# Autodesk Inventor assembly: Inverse belt reducer
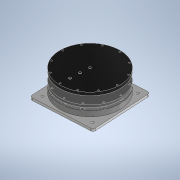
[picture p0: Inventor's stored thumbnail of the model, 180x180]
Saved by Autodesk Inventor 2022 (Build 260153000, 153)
## iProperties
Created: 2022-02-18
Part Number: Inverse belt reducer
Document SubType Name: Assembly
Designer: JK
Author: JK
## Documents named in this file (19)
- C:\Users\JK\Documents\Inventor\ScaraNema\Inverse timing belt reducer\Inverse belt reducer.iam
- C:\Users\JK\Documents\Inventor\ScaraNema\MOTOR_LONG.ipt
- C:\Users\JK\Documents\Inventor\ScaraNema\Inverse timing belt reducer\Motorsupport.ipt
- C:\Users\JK\Documents\Inventor\ScaraNema\Inverse timing belt reducer\RoboDigg GT2 16 pulley.ipt
- C:\Users\JK\Documents\Inventor\ScaraNema\Inverse timing belt reducer\M3x8SinkBolt.ipt
- C:\Users\JK\Documents\Inventor\ScaraNema\Inverse timing belt reducer\3dp idle pulley.iam
- C:\Users\JK\Documents\Inventor\ScaraNema\Inverse timing belt reducer\GT2-16 Idle pulley.iam
- C:\Users\JK\Documents\Inventor\ScaraNema\Inverse timing belt reducer\spacer.ipt
- C:\Users\JK\Documents\Inventor\ScaraNema\Inverse timing belt reducer\top.ipt
- C:\Users\JK\Documents\Inventor\ScaraNema\Inverse timing belt reducer\spacer2.ipt
- C:\Users\JK\Documents\Inventor\ScaraNema\Inverse timing belt reducer\M3 washer.ipt
- C:\Users\JK\Documents\Inventor\ScaraNema\Inverse timing belt reducer\M3Nut.ipt
- C:\Users\JK\Documents\Inventor\ScaraNema\Inverse timing belt reducer\M3x20SocketBolt.ipt
- C:\Users\JK\Documents\Inventor\ScaraNema\Inverse timing belt reducer\Platform.ipt
- C:\Users\JK\Documents\Inventor\ScaraNema\Inverse timing belt reducer\r40.iam
- C:\Users\JK\Documents\Inventor\ScaraNema\Inverse timing belt reducer\Chasis.ipt
- C:\Users\JK\Documents\Inventor\ScaraNema\Base.ipt
- C:\Users\JK\Documents\Inventor\ScaraNema\Inverse timing belt reducer\122belt.ipt
- C:\Users\JK\Documents\Inventor\ScaraNema\Inverse timing belt reducer\123.ipt
## Components (39 placed, 18 different names)
1. MOTOR_LONG:1 — Coincidencia:1, Coincidencia:2, Coincidencia:3, Ángulo:2, Coincidencia:31
2. Motorsupport:1 — Coincidencia:1, Coincidencia:2, Nivelación:1, Coincidencia:6, Coincidencia:7, Ángulo:1, Ángulo:2, Coincidencia:10, Coincidencia:14, Coincidencia:20, Coincidencia:21, Coincidencia:38, Coincidencia:51
3. RoboDigg GT2 16 pulley:1 — Coincidencia:3, Nivelación:2
4. GT2-16 Idle pulley:1 [sub-assembly] — Ángulo:1, Nivelación:3, Coincidencia:9, Coincidencia:15
5. spacer:1 — Coincidencia:9, Coincidencia:10, Coincidencia:19
6. top:1 — Coincidencia:12, Coincidencia:13, Coincidencia:14, Coincidencia:16, Coincidencia:18, Coincidencia:23, Coincidencia:24, Coincidencia:31
7. spacer2:1 — Coincidencia:15, Coincidencia:16, Coincidencia:17
8. M3 washer:1 — Coincidencia:17, Coincidencia:18, Coincidencia:25, Coincidencia:26
9. M3 washer:2 — Coincidencia:19, Coincidencia:20
10. M3x20SocketBolt:7 — Coincidencia:25, Coincidencia:26
11. Platform:1 — Coincidencia:46
12. r40:1 [sub-assembly] — Coincidencia:36, Nivelación:4, Coincidencia:40, Coincidencia:41, Coincidencia:44, Coincidencia:45, Coincidencia:46, Coincidencia:47, Coincidencia:48, Coincidencia:52, Coincidencia:53
13. Chasis:1 — Coincidencia:36, Coincidencia:38, Coincidencia:49, Coincidencia:50
14. M3x20SocketBolt:8 — Coincidencia:40, Coincidencia:41
15. Base:1 — Coincidencia:44, Coincidencia:49, Coincidencia:50
16. 122belt:1 — Coincidencia:45, Coincidencia:47, Coincidencia:48
17. 123:1 — Coincidencia:51, Coincidencia:52, Coincidencia:53
18. M3x8SinkBolt:1 — Nivelación:1
19. M3x8SinkBolt:2
20. M3x8SinkBolt:3
21. M3x8SinkBolt:4
22. 3dp idle pulley:1 [sub-assembly] — Coincidencia:6, Coincidencia:7, Nivelación:2, Nivelación:4
23. 3dp idle pulley:2 [sub-assembly]
24. 3dp idle pulley:3 [sub-assembly]
25. 3dp idle pulley:4 [sub-assembly]
26. 3dp idle pulley:5 [sub-assembly] — Coincidencia:13
27. 3dp idle pulley:6 [sub-assembly] — Nivelación:3, Coincidencia:12
28. M3x20SocketBolt:1 — Coincidencia:23, Coincidencia:24
29. M3Nut:1 — Coincidencia:21
30. M3x20SocketBolt:2
31. M3Nut:2
32. M3x20SocketBolt:3
33. M3Nut:3
34. M3x20SocketBolt:4
35. M3Nut:4
36. M3x20SocketBolt:5
37. M3Nut:5
38. M3x20SocketBolt:6
39. M3Nut:6
## Component patterns: (4 elements, first: M3x8SinkBolt:1), (6 elements, first: 3dp idle pulley:1), (6 elements, first: M3x20SocketBolt:1 + M3Nut:1)
## Relationships (42: Mate 36, Flush 4, Angle 2)
- Coincidencia:1 [Mate]: MOTOR_LONG:1 ↔ Motorsupport:1
- Coincidencia:2 [Mate]: MOTOR_LONG:1 ↔ Motorsupport:1
- Coincidencia:3 [Mate]: MOTOR_LONG:1 ↔ RoboDigg GT2 16 pulley:1
- Nivelación:1 [Flush]: Motorsupport:1 ↔ M3x8SinkBolt:1
- Coincidencia:6 [Mate]: Motorsupport:1 ↔ 3dp idle pulley:1
- Coincidencia:7 [Mate]: Motorsupport:1 ↔ 3dp idle pulley:1
- Nivelación:2 [Flush]: RoboDigg GT2 16 pulley:1 ↔ 3dp idle pulley:1
- Ángulo:1 [Angle] (0 deg): Motorsupport:1 ↔ GT2-16 Idle pulley:1
- Ángulo:2 [Angle] (0 deg): MOTOR_LONG:1 ↔ Motorsupport:1
- Nivelación:3 [Flush]: GT2-16 Idle pulley:1 ↔ 3dp idle pulley:6
- Coincidencia:9 [Mate]: GT2-16 Idle pulley:1 ↔ spacer:1
- Coincidencia:10 [Mate]: Motorsupport:1 ↔ spacer:1
- Coincidencia:12 [Mate]: top:1 ↔ 3dp idle pulley:6
- Coincidencia:13 [Mate]: top:1 ↔ 3dp idle pulley:5
- Coincidencia:14 [Mate]: Motorsupport:1 ↔ top:1
- Coincidencia:15 [Mate]: GT2-16 Idle pulley:1 ↔ spacer2:1
- Coincidencia:16 [Mate]: top:1 ↔ spacer2:1
- Coincidencia:17 [Mate]: spacer2:1 ↔ M3 washer:1
- Coincidencia:18 [Mate]: top:1 ↔ M3 washer:1
- Coincidencia:19 [Mate]: spacer:1 ↔ M3 washer:2
- Coincidencia:20 [Mate]: Motorsupport:1 ↔ M3 washer:2
- Coincidencia:21 [Mate]: Motorsupport:1 ↔ M3Nut:1
- Coincidencia:23 [Mate]: top:1 ↔ M3x20SocketBolt:1
- Coincidencia:24 [Mate]: top:1 ↔ M3x20SocketBolt:1
- Coincidencia:25 [Mate]: M3 washer:1 ↔ M3x20SocketBolt:7
- Coincidencia:26 [Mate]: M3 washer:1 ↔ M3x20SocketBolt:7
- Coincidencia:31 [Mate]: MOTOR_LONG:1 ↔ top:1
- Coincidencia:36 [Mate]: r40:1 ↔ Chasis:1
- Coincidencia:38 [Mate]: Motorsupport:1 ↔ Chasis:1
- Nivelación:4 [Flush] (4 mm): r40:1 ↔ 3dp idle pulley:1
- Coincidencia:40 [Mate]: r40:1 ↔ M3x20SocketBolt:8
- Coincidencia:41 [Mate]: r40:1 ↔ M3x20SocketBolt:8
- Coincidencia:44 [Mate]: r40:1 ↔ Base:1
- Coincidencia:45 [Mate]: r40:1 ↔ 122belt:1
- Coincidencia:46 [Mate]: Platform:1 ↔ r40:1
- Coincidencia:47 [Mate]: r40:1 ↔ 122belt:1
- Coincidencia:48 [Mate]: r40:1 ↔ 122belt:1
- Coincidencia:49 [Mate]: Chasis:1 ↔ Base:1
- Coincidencia:50 [Mate]: Chasis:1 ↔ Base:1
- Coincidencia:51 [Mate]: Motorsupport:1 ↔ 123:1
- Coincidencia:52 [Mate]: r40:1 ↔ 123:1
- Coincidencia:53 [Mate]: r40:1 ↔ 123:1
